# Autodesk Inventor assembly: RadioPanelMount
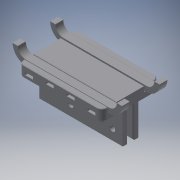
[picture p0: Inventor's stored thumbnail of the model, 180x180]
Saved by Autodesk Inventor 2018 (Build 220112000, 112)
## iProperties
Created: 2017-09-08
Part Number: RadioPanelMount
Document SubType Name: Assembly
Designer: Srinity
Author: Srinity
## Documents named in this file (3)
- C:\Users\Srinity\Documents\DIY Projects\ModularFRCPlatform\RadioPanelMount.iam
- C:\Users\Srinity\Documents\DIY Projects\ModularFRCPlatform\RadioPanelMountA.ipt
- C:\Users\Srinity\Documents\DIY Projects\ModularFRCPlatform\RadioPanelMountB.ipt
## Components (3 placed, 2 different names)
1. RadioPanelMountA:1 — Mate:1, Mate:2, Mate:3, Mate:4, Mate:5, Mate:6
2. RadioPanelMountB:1 — Mate:1, Mate:2, Mate:6
3. RadioPanelMountB:2 — Mate:3, Mate:4, Mate:5
## Relationships (6: Mate 6)
- Mate:1 (3.175 mm): RadioPanelMountA:1 ↔ RadioPanelMountB:1
- Mate:2: RadioPanelMountA:1 ↔ RadioPanelMountB:1
- Mate:3 (3.175 mm): RadioPanelMountA:1 ↔ RadioPanelMountB:2
- Mate:4: RadioPanelMountA:1 ↔ RadioPanelMountB:2
- Mate:5: RadioPanelMountA:1 ↔ RadioPanelMountB:2
- Mate:6: RadioPanelMountA:1 ↔ RadioPanelMountB:1
